# Autodesk Inventor assembly: Holder
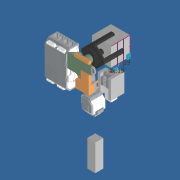
[picture p0: Inventor's stored thumbnail of the model, 180x180]
Saved by Autodesk Inventor 2020 (Build 240168000, 168)
## iProperties
Created: 2019-12-14
Part Number: Holder
Document SubType Name: Assembly
Designer: Jack
Author: Jack
## Documents named in this file (12)
- D:\Code\Python\EV3_Cuber\3D Model\Holder.iam
- D:\Code\Python\EV3_Cuber\3D Model\HolderGear.ipt
- D:\Code\Python\EV3_Cuber\3D Model\HolderShaft.ipt
- D:\Code\Python\EV3_Cuber\3D Model\Cube.ipt
- D:\Code\Python\EV3_Cuber\3D Model\Hand.ipt
- D:\Code\Python\EV3_Cuber\3D Model\MotorL.ipt
- D:\Code\Python\EV3_Cuber\3D Model\Brick.ipt
- D:\Code\Python\EV3_Cuber\3D Model\Gear 24.ipt
- D:\Code\Python\EV3_Cuber\3D Model\MotorHolder_Y.ipt
- D:\Code\Python\EV3_Cuber\3D Model\MotorM.ipt
- D:\Code\Python\EV3_Cuber\3D Model\MotorRail.ipt
- D:\Code\Python\EV3_Cuber\3D Model\MotorHolder_X.ipt
## Components (11 placed, 11 different names)
1. HolderShaft:1 — Mate:8, Mate:9, Mate:10, Angle:4, Rotational:3, Mate:13, Flush:2, Mate:14
2. HolderGear:1 — Angle:1, Angle:2, Mate:5, Mate:7, Flush:1, Rotational:3, Mate:15
3. Cube:1 — Angle:1, Angle:2, Mate:5, Mate:7, Angle:3, Mate:11, Mate:15, Flush:3, Mate:16
4. Hand:1 — Angle:3, Mate:11, Rigid:1, Flush:3, Mate:16
5. MotorL:1 — Rotational:2, Mate:10, Angle:4
6. Brick:1 — Mate:8, Mate:9
7. Gear 24:1 — Rotational:2, Flush:1
8. MotorHolder_Y:1 — Mate:13, Flush:2, Mate:14, Angle:5
9. MotorM:1 — Rigid:1, Angle:5, Mate:17, Mate:18, Flush:4
10. MotorRail:1
11. MotorHolder_X:1 — Mate:17, Mate:18, Flush:4
## Relationships (24: Mate 12, Angle 5, Flush 4, RevoluteJoint 2, WeldJoint 1)
- Angle:1 (0 deg): HolderGear:1 ↔ Cube:1
- Angle:2 (0 deg): HolderGear:1 ↔ Cube:1
- Mate:5 (0.5 mm): HolderGear:1 ↔ Cube:1
- Mate:7 (0.5 mm): HolderGear:1 ↔ Cube:1
- Mate:8: HolderShaft:1 ↔ Brick:1
- Mate:9: HolderShaft:1 ↔ Brick:1
- Rotational:2 [RevoluteJoint]: MotorL:1 ↔ Gear 24:1
- Flush:1: HolderGear:1 ↔ Gear 24:1
- Mate:10: HolderShaft:1 ↔ MotorL:1
- Angle:3 (0 deg): Cube:1 ↔ Hand:1
- Mate:11 (0.5 mm): Cube:1 ↔ Hand:1
- Angle:4 (0 deg): HolderShaft:1 ↔ MotorL:1
- Rotational:3 [RevoluteJoint]: HolderShaft:1 ↔ HolderGear:1
- Mate:13 (0.2 mm): HolderShaft:1 ↔ MotorHolder_Y:1
- Flush:2: HolderShaft:1 ↔ MotorHolder_Y:1
- Mate:14 (0.2 mm): HolderShaft:1 ↔ MotorHolder_Y:1
- Mate:15: HolderGear:1 ↔ Cube:1
- Rigid:1 [WeldJoint] (-8 mm): Hand:1 ↔ MotorM:1
- Angle:5 (0 deg): MotorHolder_Y:1 ↔ MotorM:1
- Flush:3 (24.5 mm): Cube:1 ↔ Hand:1
- Mate:16: Cube:1 ↔ Hand:1
- Mate:17 (0.2 mm): MotorM:1 ↔ MotorHolder_X:1
- Mate:18 (0.2 mm): MotorM:1 ↔ MotorHolder_X:1
- Flush:4: MotorM:1 ↔ MotorHolder_X:1
